# Autodesk Inventor assembly: Main Body with Arduino and Gyro Mounts
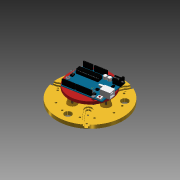
[picture p0: Inventor's stored thumbnail of the model, 180x180]
Saved by Autodesk Inventor 2014 (Build 180170000, 170)
## iProperties
Created: 2014-02-14
Part Number: Main Body with Arduino and Gyro Mounts
Document SubType Name: Assembly
Designer: Spooner
Author: Spooner
## Documents named in this file (9)
- C:\Users\Spooner\Documents\Inventor\FerretBall Robot\3Pod\Inventor 2014 Files\Main Body with Arduino and Gyro Mounts.iam
- C:\Users\Spooner\Documents\Inventor\FerretBall Robot\3Pod\Inventor 2014 Files\Arduino Mount.ipt
- C:\Users\Spooner\Documents\Inventor\FerretBall Robot\3Pod\Inventor 2014 Files\Body.ipt
- C:\Users\Spooner\Documents\Inventor\FerretBall Robot\3Pod\Inventor 2014 Files\Gyro Mount.ipt
- C:\Users\Spooner\Documents\Inventor\FerretBall Robot\3Pod\Inventor 2014 Files\Offset.ipt
- C:\Users\Spooner\Documents\Inventor\Content Center Files\R2014\en-US\JIS B 1111(1)\JIS B 1111 - M3x30(1).ipt
- C:\Users\Spooner\Documents\Inventor\Content Center Files\R2014\en-US\JIS B 1181 U\JIS B 1181 - B M3.ipt
- C:\Users\Spooner\Documents\Inventor\FerretBall Robot\3Pod\Inventor 2014 Files\Arduino.ipt
- C:\Users\Spooner\Documents\Inventor\Content Center Files\R2014\en-US\JIS B 1111(1)\JIS B 1111 - M3x12(1).ipt
## Components (21 placed, 8 different names)
1. Arduino Mount:1 — Insert:6, Insert:7, Insert:8, Insert:9, Insert:10, Insert:14, Mate:1, Insert:19, Insert:20, Insert:21, Insert:22
2. Body:1 — Insert:1, Insert:2, Insert:3, Insert:11, Insert:12, Insert:13
3. Gyro Mount:1 — Insert:4, Insert:5, Insert:6, Insert:7
4. Offset:1 — Insert:3, Insert:5
5. Offset:2 — Insert:2, Insert:4
6. Offset:3 — Insert:1
7. JIS B 1111 M3x30:4 — Insert:8
8. JIS B 1111 M3x30:2 — Insert:9
9. JIS B 1111 M3x30:3 — Insert:10
10. JIS B 1181 (unchamfered) - Metric B M3:1 — Insert:11
11. JIS B 1181 (unchamfered) - Metric B M3:2 — Insert:12
12. JIS B 1181 (unchamfered) - Metric B M3:3 — Insert:13
13. Arduino:1 — Insert:14, Mate:1, Insert:15, Insert:16, Insert:17, Insert:18
14. JIS B 1111 M3x12:3 — Insert:15
15. JIS B 1111 M3x12:1 — Insert:18
16. JIS B 1111 M3x12:2 — Insert:16
17. JIS B 1111 M3x12:4 — Insert:17
18. JIS B 1181 (unchamfered) - Metric B M3:4 — Insert:22
19. JIS B 1181 (unchamfered) - Metric B M3:5 — Insert:21
20. JIS B 1181 (unchamfered) - Metric B M3:6 — Insert:20
21. JIS B 1181 (unchamfered) - Metric B M3:7 — Insert:19
## Relationships (23: Insert 22, Mate 1)
- Insert:1: Body:1 ↔ Offset:3
- Insert:2: Body:1 ↔ Offset:2
- Insert:3: Body:1 ↔ Offset:1
- Insert:4: Gyro Mount:1 ↔ Offset:2
- Insert:5: Gyro Mount:1 ↔ Offset:1
- Insert:6: Arduino Mount:1 ↔ Gyro Mount:1
- Insert:7: Arduino Mount:1 ↔ Gyro Mount:1
- Insert:8: Arduino Mount:1 ↔ JIS B 1111 M3x30:4
- Insert:9: Arduino Mount:1 ↔ JIS B 1111 M3x30:2
- Insert:10: Arduino Mount:1 ↔ JIS B 1111 M3x30:3
- Insert:11: Body:1 ↔ JIS B 1181 (unchamfered) - Metric B M3:1
- Insert:12: Body:1 ↔ JIS B 1181 (unchamfered) - Metric B M3:2
- Insert:13: Body:1 ↔ JIS B 1181 (unchamfered) - Metric B M3:3
- Insert:14: Arduino Mount:1 ↔ Arduino:1
- Mate:1: Arduino Mount:1 ↔ Arduino:1
- Insert:15: Arduino:1 ↔ JIS B 1111 M3x12:3
- Insert:16: Arduino:1 ↔ JIS B 1111 M3x12:2
- Insert:17: Arduino:1 ↔ JIS B 1111 M3x12:4
- Insert:18: Arduino:1 ↔ JIS B 1111 M3x12:1
- Insert:19: Arduino Mount:1 ↔ JIS B 1181 (unchamfered) - Metric B M3:7
- Insert:20: Arduino Mount:1 ↔ JIS B 1181 (unchamfered) - Metric B M3:6
- Insert:21: Arduino Mount:1 ↔ JIS B 1181 (unchamfered) - Metric B M3:5
- Insert:22: Arduino Mount:1 ↔ JIS B 1181 (unchamfered) - Metric B M3:4
